# Autodesk Inventor assembly: Assembly6
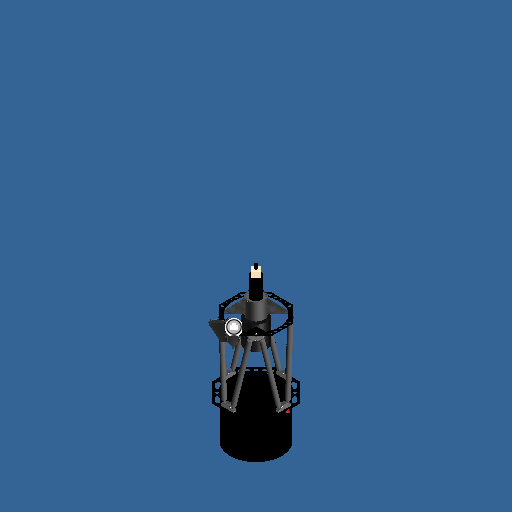
[picture p0: Inventor's stored thumbnail of the model, 512x512]
Saved by Autodesk Inventor 2026.2 (Build 302298000, 298)
## iProperties
Created: 2025-12-09
Part Number: Assembly6
Document SubType Name: Assembly
Designer: Thoma
Mass: 27295.5 g
Surface Area: 25498 cm^2
Volume: 10830.6 cm^3
Density: 2.52023 g/cm^3
Author: Thoma
## Documents named in this file (32)
- C:\Users\Thoma\OneDrive\Desktop\dir\telescope_cover\main\version_2\Main_v4.iam
- C:\Users\Thoma\OneDrive\Desktop\dir\telescope_cover\telescope\version_3\Telescope_End.ipt
- C:\Users\Thoma\OneDrive\Desktop\dir\telescope_cover\telescope\version_3\Triangle.ipt
- C:\Users\Thoma\OneDrive\Desktop\dir\telescope_cover\telescope\version_3\Triangle_Bracket_Top.ipt
- C:\Users\Thoma\OneDrive\Desktop\dir\telescope_cover\telescope\version_3\Carbon_Fibre.ipt
- C:\Users\Thoma\OneDrive\Desktop\dir\telescope_cover\telescope\version_3\5mm Screw.ipt
- C:\Users\Thoma\OneDrive\Desktop\dir\telescope_cover\telescope\version_3\35mm_bolt.ipt
- C:\Users\Thoma\OneDrive\Desktop\dir\telescope_cover\telescope\version_3\Triangle_Bracket_Bottom_MIR.ipt
- C:\Users\Thoma\OneDrive\Desktop\dir\telescope_cover\telescope\version_3\Telescope_Base.ipt
- C:\Users\Thoma\OneDrive\Desktop\dir\telescope_cover\telescope\version_3\Full_shaft_Simplify_3.ipt
- C:\Users\Thoma\OneDrive\Desktop\dir\telescope_cover\telescope\version_3\30mm_bolt.ipt
- C:\Users\Thoma\OneDrive\Desktop\dir\telescope_cover\telescope\version_3\Baffle.ipt
- C:\Users\Thoma\OneDrive\Desktop\dir\telescope_cover\telescope\version_3\Bottom_End_Top.ipt
- C:\Users\Thoma\OneDrive\Desktop\dir\telescope_cover\telescope\version_3\Laser.ipt
- C:\Users\Thoma\OneDrive\Desktop\dir\telescope_cover\cover\central_cover_v1.ipt
- C:\Users\Thoma\OneDrive\Desktop\dir\telescope_cover\cover\base_plate_v11.ipt
- C:\Users\Thoma\OneDrive\Desktop\dir\telescope_cover\cover\base_plate_bottom_v5.ipt
- C:\Users\Thoma\OneDrive\Documents\Inventor\Content Center Files\R2026\en-US\ISO 7089\ISO 7089 - 4 - 140 HV(1).ipt
- C:\Users\Thoma\OneDrive\Documents\Inventor\Content Center Files\R2026\en-US\ISO 4762(2)\ISO 4762 - M4 x 25ISO.ipt
- C:\Users\Thoma\OneDrive\Documents\Inventor\Content Center Files\R2026\en-US\ISO 4035(2)\ISO 4035 - M4 - ISO.ipt
- C:\Users\Thoma\OneDrive\Desktop\dir\telescope_cover\servo\DSS-M15S Servo.ipt
- C:\Users\Thoma\OneDrive\Documents\Inventor\Content Center Files\R2026\en-US\ISO 4762(2)\ISO 4762 - M4 x 16ISO.ipt
- C:\Users\Thoma\OneDrive\Desktop\dir\telescope_cover\cover\pawn_v3.ipt
- C:\Users\Thoma\OneDrive\Documents\Inventor\Content Center Files\R2026\en-US\DIN 6796\DIN 6796 - 2.ipt
- C:\Users\Thoma\OneDrive\Documents\Inventor\Content Center Files\R2026\en-US\DIN 912\DIN 912 - M2 x 0.4 x 8 x 7.ipt
- C:\Users\Thoma\OneDrive\Documents\Inventor\Content Center Files\R2026\en-US\DIN 912\DIN 912 - M2 x 0.4 x 5 x 4.ipt
- C:\Users\Thoma\OneDrive\Desktop\dir\telescope_cover\cover\rod_v11.ipt
- C:\Users\Thoma\OneDrive\Documents\Inventor\Content Center Files\R2026\en-US\ISO 7092\ISO 7092 - ST 4 - 140 HV.ipt
- C:\Users\Thoma\OneDrive\Desktop\dir\telescope_cover\cover\Cover_Upper_v5.ipt
- C:\Users\Thoma\OneDrive\Desktop\dir\telescope_cover\cover\4mm_washer_1mm.ipt
- C:\Users\Thoma\OneDrive\Documents\Inventor\Content Center Files\R2026\en-US\ISO 4762(2)\ISO 4762 - M4 x 20ISO.ipt
- C:\Users\Thoma\OneDrive\Desktop\dir\telescope_cover\servo\Limit Switch v3\Limit Switch v3\Limit Switch v3.ipt
## Components (98 placed, 31 different names)
1. base_plate_v11:1 — Mate:229, Angle:85, Mate:230, Mate:231, Mate:233, Mate:234, Mate:239, Mate:240, Mate:241, Angle:88, Mate:243, Mate:244, Mate:245, Angle:91, Mate:247, Mate:248, Mate:249, Angle:92, Mate:262, Mate:263, Mate:264, Mate:271, Mate:272, Mate:273, Mate:274, Mate:275, Mate:276, Mate:277, Mate:278, Mate:282, Mate:307, Mate:308, Mate:309, Mate:310, Mate:312, Mate:314
2. base_plate_bottom_v5:1 — Mate:232, Mate:233, Mate:234, Mate:242, Angle:89, Mate:246, Angle:90, Mate:250, Flush:227, Flush:228, Angle:93
3. ISO 7089 4:2 — Mate:239, Mate:240, Insert:2
4. ISO 4762 M4 x 25:1 — Insert:2, Angle:88
5. ISO 4035 M4:1 — Mate:241, Mate:242, Angle:89
6. ISO 7089 4:3 — Mate:243, Mate:244, Insert:3
7. ISO 4762 M4 x 16:1 — Insert:3, Angle:91
8. ISO 4035 M4:2 — Mate:245, Mate:246, Angle:90
9. ISO 7089 4:4 — Mate:247, Mate:248, Insert:4
10. ISO 4762 M4 x 16:2 — Insert:4
11. ISO 4035 M4:3 — Mate:249, Mate:250, Angle:93
12. pawn_v3:1 — Angle:92, Mate:281, Mate:282, Mate:311, Mate:313
13. DSS-M15S Servo:1 — Mate:262, Mate:263, Mate:264, Mate:279, Mate:280
14. DIN 6796 2:1 — Mate:271, Mate:272, Insert:6
15. DIN 912 - replaced by DIN EN ISO 4762 M2 x 8:1 — Insert:6
16. DIN 6796 2:2 — Mate:273, Mate:274, Insert:7
17. DIN 912 - replaced by DIN EN ISO 4762 M2 x 5:1 — Insert:7
18. DIN 6796 2:3 — Mate:275, Mate:276, Insert:8
19. DIN 912 - replaced by DIN EN ISO 4762 M2 x 8:2 — Insert:8
20. DIN 6796 2:4 — Mate:277, Mate:278, Insert:9
21. DIN 912 - replaced by DIN EN ISO 4762 M2 x 8:3 — Insert:9
22. rod_v11:1 — Mate:279, Mate:280, Mate:281, Mate:287, Mate:288, Tangent:34, Mate:289, Mate:290, Mate:291, Mate:292, Mate:293, Mate:294, Mate:295, Mate:297, Mate:298, Mate:299, Mate:301, Mate:302, Mate:303, Mate:305, Mate:306, Mate:315
23. Cover_Upper_v5:1 — Mate:287, Mate:288, Tangent:34, Mate:296, Mate:300, Mate:304
24. 4mm_washer_1mm:1 — Mate:289, Mate:294
25. 4mm_washer_1mm:2 — Mate:290, Mate:293
26. 4mm_washer_1mm:3 — Mate:291, Mate:292
27. ISO 7092 ST 4 - 140 HV:3 — Mate:295, Mate:296, Insert:12
28. ISO 4762 M4 x 16:3 — Insert:12
29. ISO 7092 ST 4 - 140 HV:4 — Mate:297, Mate:298, Insert:13
30. ISO 4035 M4:5 — Insert:13
31. ISO 7092 ST 4 - 140 HV:5 — Mate:299, Mate:300, Insert:14
32. ISO 4762 M4 x 16:4 — Insert:14
33. ISO 7092 ST 4 - 140 HV:6 — Mate:301, Mate:302, Insert:15
34. ISO 4035 M4:6 — Insert:15
35. ISO 7092 ST 4 - 140 HV:7 — Mate:303, Mate:304, Insert:16
36. ISO 4762 M4 x 16:5 — Insert:16
37. ISO 7092 ST 4 - 140 HV:8 — Mate:305, Mate:306, Insert:17
38. ISO 4035 M4:7 — Insert:17
39. ISO 4762 M4 x 20:1 — Mate:307, Mate:308
40. ISO 4035 M4:8 — Mate:309, Mate:310
41. ISO 4762 M4 x 20:2 — Mate:311, Mate:312
42. ISO 4035 M4:9 — Mate:313, Mate:314
43. Limit Switch v3:1 — Tangent:35
44. Limit Switch v3:2 — Flush:227, Flush:228, Mate:315
45. Laser:2 — Mate:214, Flush:220, Flush:221
46. Laser:1 — Mate:215, Flush:218, Flush:219
47. Baffle:1 — Mate:83
48. Carbon_Fibre:1 — Mate:7, Mate:11, Flush:1, Mate:12, Mate:13, Mate:14, Mate:15, Mate:62, Mate:83, Mate:92, Mate:93, Mate:96, Mate:97, Mate:98, Mate:100, Mate:123, Mate:124, Mate:125, Mate:213, Mate:220, Angle:84, Flush:223, Flush:224, Flush:225, Flush:226
49. Telescope_Base:1 — Mate:62, Angle:31, Mate:89, Mate:90, Angle:40, Mate:108, Mate:109, Angle:48, Mate:110, Mate:111, Angle:49, Mate:112, Mate:113, Angle:50, Mate:214, Mate:215, Flush:218, Flush:221
50. Telescope_End:1 — Mate:1, Mate:2, Angle:2, Mate:7, Mate:54, Mate:55, Angle:26, Angle:31, Mate:86, Mate:88, Mate:91, Angle:41, Mate:101, Angle:45, Angle:46, Mate:114, Mate:115, Angle:51, Mate:116, Mate:117, Angle:52, Mate:118, Mate:119, Angle:53, Mate:229, Angle:85, Mate:230, Mate:231, Mate:232
51. 30mm_bolt:9 — Mate:217, Mate:218, Angle:83
52. 30mm_bolt:10 — Mate:216, Mate:219, Angle:82
53. Triangle_Bracket_Top:5 — Mate:116, Mate:117, Angle:52, Mate:129, Flush:110, Angle:60
54. Triangle_Bracket_Top:4 — Mate:101, Angle:45, Angle:46, Mate:104, Mate:105, Mate:106, Flush:103, Angle:47
55. Triangle_Bracket_Top:3 — Mate:86, Mate:88, Mate:94, Angle:54, Angle:55, Mate:122, Flush:106, Angle:56
56. Triangle_Bracket_Top:1 — Mate:1, Mate:2, Angle:2, Mate:8, Mate:9, Angle:4, Mate:47, Angle:22, Mate:58
57. 5mm Screw:14 — Mate:220, Flush:222, Angle:84
58. Triangle:1 — Mate:8, Mate:9, Angle:4, Mate:11, Flush:1, Angle:5, Angle:6, Mate:46, Mate:222, Mate:223
59. Triangle:5 — Mate:92, Mate:93, Mate:94, Mate:128, Flush:109, Angle:59, Flush:181, Angle:81, Mate:225, Mate:227
60. Triangle:6 — Mate:96, Mate:97, Mate:98, Flush:102, Angle:44, Mate:104, Mate:105, Flush:222, Mate:221, Mate:228
61. Triangle:7 — Mate:123, Mate:124, Mate:125, Mate:126, Flush:107, Angle:57, Mate:127, Flush:108, Angle:58, Mate:224, Mate:226
62. 35mm_bolt:6 — Mate:122, Flush:106, Angle:56
63. 35mm_bolt:7 — Mate:129, Flush:110, Angle:60
64. 35mm_bolt:4 — Mate:46, Mate:47, Angle:22
65. 35mm_bolt:5 — Mate:106, Flush:103, Angle:47
66. 5mm Screw:9 — Mate:100, Flush:102, Angle:44
67. 5mm Screw:13 — Mate:213, Flush:181, Angle:81
68. 5mm Screw:10 — Mate:126, Flush:107, Angle:57
69. 5mm Screw:2 — Mate:14, Mate:15, Angle:6
70. 5mm Screw:1 — Mate:12, Mate:13, Angle:5
71. 5mm Screw:11 — Mate:127, Flush:108, Angle:58
72. 5mm Screw:12 — Mate:128, Flush:109, Angle:59
73. Full_shaft_Simplify_3:1
74. Full_shaft_Simplify_3:2 — Tangent:26
75. Full_shaft_Simplify_3:3
76. Full_shaft_Simplify_3:4
77. Full_shaft_Simplify_3:5
78. Full_shaft_Simplify_3:6
79. Full_shaft_Simplify_3:7
80. Full_shaft_Simplify_3:8 — Tangent:31, Tangent:33
81. 30mm_bolt:7 — Mate:120, Flush:104, Angle:54
82. 30mm_bolt:1 — Mate:121, Flush:105, Angle:55
83. 30mm_bolt:8 — Mate:80, Flush:13, Angle:39
84. 30mm_bolt:6 — Mate:78, Flush:11, Angle:37
85. 30mm_bolt:3 — Mate:79, Flush:12, Angle:38
86. 30mm_bolt:2 — Mate:77, Flush:10, Angle:36
87. Triangle_Bracket_Bottom_MIR:4 — Mate:118, Mate:119, Angle:53, Mate:216, Mate:217, Mate:218, Mate:219, Angle:82, Angle:83
88. Triangle_Bracket_Bottom_MIR:3 — Mate:114, Mate:115, Angle:51, Mate:120, Flush:104, Mate:121, Flush:105
89. Triangle_Bracket_Bottom_MIR:2 — Mate:55, Mate:58, Angle:26, Mate:77, Flush:10, Angle:36, Mate:78, Flush:11, Angle:37, Tangent:31
90. Triangle_Bracket_Bottom_MIR:1 — Mate:54, Mate:79, Flush:12, Angle:38, Mate:80, Flush:13, Angle:39, Mate:91, Angle:41
91. Bottom_End_Top:4 — Mate:112, Mate:113, Angle:50, Tangent:26, Tangent:33
92. Bottom_End_Top:3 — Mate:110, Mate:111, Angle:49, Flush:219
93. Bottom_End_Top:2 — Mate:108, Mate:109, Angle:48
94. Bottom_End_Top:1 — Mate:89, Mate:90, Angle:40, Flush:220
95. central_cover_v1:1 — Mate:221, Mate:222, Flush:223, Tangent:35
96. central_cover_v1:2 — Mate:223, Mate:224, Flush:224
97. central_cover_v1:3 — Mate:225, Mate:226, Flush:225
98. central_cover_v1:4 — Mate:227, Mate:228, Flush:226
## Relationships (222: Mate 137, Angle 41, Flush 26, Insert 13, Tangent 5)
- Mate:1: Telescope_End:1 ↔ Triangle_Bracket_Top:1
- Mate:2: Telescope_End:1 ↔ Triangle_Bracket_Top:1
- Angle:2 (0 deg): Telescope_End:1 ↔ Triangle_Bracket_Top:1
- Mate:7: Carbon_Fibre:1 ↔ Telescope_End:1
- Mate:8: Triangle_Bracket_Top:1 ↔ Triangle:1
- Mate:9: Triangle_Bracket_Top:1 ↔ Triangle:1
- Angle:4 (0 deg): Triangle_Bracket_Top:1 ↔ Triangle:1
- Mate:11: Carbon_Fibre:1 ↔ Triangle:1
- Flush:1: Carbon_Fibre:1 ↔ Triangle:1
- Mate:12: Carbon_Fibre:1 ↔ 5mm Screw:1
- Mate:13: Carbon_Fibre:1 ↔ 5mm Screw:1
- Angle:5 (0 deg): Triangle:1 ↔ 5mm Screw:1
- Mate:14: Carbon_Fibre:1 ↔ 5mm Screw:2
- Mate:15: Carbon_Fibre:1 ↔ 5mm Screw:2
- Angle:6 (0 deg): Triangle:1 ↔ 5mm Screw:2
- Mate:46: Triangle:1 ↔ 35mm_bolt:4
- Mate:47: Triangle_Bracket_Top:1 ↔ 35mm_bolt:4
- Angle:22 (0 deg): Triangle_Bracket_Top:1 ↔ 35mm_bolt:4
- Mate:54: Telescope_End:1 ↔ Triangle_Bracket_Bottom_MIR:1
- Mate:55: Telescope_End:1 ↔ Triangle_Bracket_Bottom_MIR:2
- Mate:58: Triangle_Bracket_Top:1 ↔ Triangle_Bracket_Bottom_MIR:2
- Angle:26 (0 deg): Telescope_End:1 ↔ Triangle_Bracket_Bottom_MIR:2
- Mate:62: Carbon_Fibre:1 ↔ Telescope_Base:1
- Angle:31 (0 deg): Telescope_Base:1 ↔ Telescope_End:1
- Mate:77: 30mm_bolt:2 ↔ Triangle_Bracket_Bottom_MIR:2
- Flush:10: 30mm_bolt:2 ↔ Triangle_Bracket_Bottom_MIR:2
- Angle:36 (0 deg): 30mm_bolt:2 ↔ Triangle_Bracket_Bottom_MIR:2
- Mate:78: 30mm_bolt:6 ↔ Triangle_Bracket_Bottom_MIR:2
- Flush:11: 30mm_bolt:6 ↔ Triangle_Bracket_Bottom_MIR:2
- Angle:37 (0 deg): 30mm_bolt:6 ↔ Triangle_Bracket_Bottom_MIR:2
- Mate:79: 30mm_bolt:3 ↔ Triangle_Bracket_Bottom_MIR:1
- Flush:12: 30mm_bolt:3 ↔ Triangle_Bracket_Bottom_MIR:1
- Angle:38 (0 deg): 30mm_bolt:3 ↔ Triangle_Bracket_Bottom_MIR:1
- Mate:80: 30mm_bolt:8 ↔ Triangle_Bracket_Bottom_MIR:1
- Flush:13: 30mm_bolt:8 ↔ Triangle_Bracket_Bottom_MIR:1
- Angle:39 (0 deg): 30mm_bolt:8 ↔ Triangle_Bracket_Bottom_MIR:1
- Mate:83: Baffle:1 ↔ Carbon_Fibre:1
- Mate:86: Telescope_End:1 ↔ Triangle_Bracket_Top:3
- Mate:88: Telescope_End:1 ↔ Triangle_Bracket_Top:3
- Mate:89: Telescope_Base:1 ↔ Bottom_End_Top:1
- Mate:90: Telescope_Base:1 ↔ Bottom_End_Top:1
- Angle:40 (0 deg): Telescope_Base:1 ↔ Bottom_End_Top:1
- Mate:91: Telescope_End:1 ↔ Triangle_Bracket_Bottom_MIR:1
- Angle:41 (0 deg): Telescope_End:1 ↔ Triangle_Bracket_Bottom_MIR:1
- Mate:92: Carbon_Fibre:1 ↔ Triangle:5
- Mate:93: Carbon_Fibre:1 ↔ Triangle:5
- Mate:94: Triangle_Bracket_Top:3 ↔ Triangle:5
- Mate:96: Carbon_Fibre:1 ↔ Triangle:6
- Mate:97: Carbon_Fibre:1 ↔ Triangle:6
- Mate:98: Carbon_Fibre:1 ↔ Triangle:6
- Mate:100: Carbon_Fibre:1 ↔ 5mm Screw:9
- Flush:102: Triangle:6 ↔ 5mm Screw:9
- Angle:44 (0 deg): Triangle:6 ↔ 5mm Screw:9
- Mate:101: Telescope_End:1 ↔ Triangle_Bracket_Top:4
- Angle:45 (0 deg): Telescope_End:1 ↔ Triangle_Bracket_Top:4
- Angle:46 (0 deg): Telescope_End:1 ↔ Triangle_Bracket_Top:4
- Mate:104: Triangle_Bracket_Top:4 ↔ Triangle:6
- Mate:105: Triangle_Bracket_Top:4 ↔ Triangle:6
- Mate:106: Triangle_Bracket_Top:4 ↔ 35mm_bolt:5
- Flush:103: Triangle_Bracket_Top:4 ↔ 35mm_bolt:5
- Angle:47 (0 deg): Triangle_Bracket_Top:4 ↔ 35mm_bolt:5
- Mate:108: Telescope_Base:1 ↔ Bottom_End_Top:2
- Mate:109: Telescope_Base:1 ↔ Bottom_End_Top:2
- Angle:48 (0 deg): Telescope_Base:1 ↔ Bottom_End_Top:2
- Mate:110: Telescope_Base:1 ↔ Bottom_End_Top:3
- Mate:111: Telescope_Base:1 ↔ Bottom_End_Top:3
- Angle:49 (0 deg): Telescope_Base:1 ↔ Bottom_End_Top:3
- Mate:112: Telescope_Base:1 ↔ Bottom_End_Top:4
- Mate:113: Telescope_Base:1 ↔ Bottom_End_Top:4
- Angle:50 (0 deg): Telescope_Base:1 ↔ Bottom_End_Top:4
- Mate:114: Telescope_End:1 ↔ Triangle_Bracket_Bottom_MIR:3
- Mate:115: Telescope_End:1 ↔ Triangle_Bracket_Bottom_MIR:3
- Angle:51 (0 deg): Telescope_End:1 ↔ Triangle_Bracket_Bottom_MIR:3
- Mate:116: Telescope_End:1 ↔ Triangle_Bracket_Top:5
- Mate:117: Telescope_End:1 ↔ Triangle_Bracket_Top:5
- Angle:52 (0 deg): Telescope_End:1 ↔ Triangle_Bracket_Top:5
- Mate:118: Telescope_End:1 ↔ Triangle_Bracket_Bottom_MIR:4
- Mate:119: Telescope_End:1 ↔ Triangle_Bracket_Bottom_MIR:4
- Angle:53 (0 deg): Telescope_End:1 ↔ Triangle_Bracket_Bottom_MIR:4
- Mate:120: 30mm_bolt:7 ↔ Triangle_Bracket_Bottom_MIR:3
- Flush:104: 30mm_bolt:7 ↔ Triangle_Bracket_Bottom_MIR:3
- Angle:54 (0 deg): Triangle_Bracket_Top:3 ↔ 30mm_bolt:7
- Mate:121: 30mm_bolt:1 ↔ Triangle_Bracket_Bottom_MIR:3
- Flush:105: 30mm_bolt:1 ↔ Triangle_Bracket_Bottom_MIR:3
- Angle:55 (0 deg): Triangle_Bracket_Top:3 ↔ 30mm_bolt:1
- Mate:122: Triangle_Bracket_Top:3 ↔ 35mm_bolt:6
- Flush:106: Triangle_Bracket_Top:3 ↔ 35mm_bolt:6
- Angle:56 (0 deg): Triangle_Bracket_Top:3 ↔ 35mm_bolt:6
- Mate:123: Carbon_Fibre:1 ↔ Triangle:7
- Mate:124: Carbon_Fibre:1 ↔ Triangle:7
- Mate:125: Carbon_Fibre:1 ↔ Triangle:7
- Mate:126: Triangle:7 ↔ 5mm Screw:10
- Flush:107: Triangle:7 ↔ 5mm Screw:10
- Angle:57 (0 deg): Triangle:7 ↔ 5mm Screw:10
- Mate:127: Triangle:7 ↔ 5mm Screw:11
- Flush:108: Triangle:7 ↔ 5mm Screw:11
- Angle:58 (0 deg): Triangle:7 ↔ 5mm Screw:11
- Mate:128: Triangle:5 ↔ 5mm Screw:12
- Flush:109: Triangle:5 ↔ 5mm Screw:12
- Angle:59 (0 deg): Triangle:5 ↔ 5mm Screw:12
- Mate:129: Triangle_Bracket_Top:5 ↔ 35mm_bolt:7
- Flush:110: Triangle_Bracket_Top:5 ↔ 35mm_bolt:7
- Angle:60 (0 deg): Triangle_Bracket_Top:5 ↔ 35mm_bolt:7
- Mate:213: Carbon_Fibre:1 ↔ 5mm Screw:13
- Flush:181: Triangle:5 ↔ 5mm Screw:13
- Angle:81 (0 deg): Triangle:5 ↔ 5mm Screw:13
- Mate:214: Laser:2 ↔ Telescope_Base:1
- Mate:215: Laser:1 ↔ Telescope_Base:1
- Flush:218: Laser:1 ↔ Telescope_Base:1
- Flush:219 (39.316 mm): Laser:1 ↔ Bottom_End_Top:3
- Flush:220 (39.316 mm): Laser:2 ↔ Bottom_End_Top:1
- Flush:221: Laser:2 ↔ Telescope_Base:1
- Tangent:26: Full_shaft_Simplify_3:2 ↔ Bottom_End_Top:4
- Tangent:31: Full_shaft_Simplify_3:8 ↔ Triangle_Bracket_Bottom_MIR:2
- Tangent:33: Full_shaft_Simplify_3:8 ↔ Bottom_End_Top:4
- Mate:216: 30mm_bolt:10 ↔ Triangle_Bracket_Bottom_MIR:4
- Mate:217: 30mm_bolt:9 ↔ Triangle_Bracket_Bottom_MIR:4
- Mate:218: 30mm_bolt:9 ↔ Triangle_Bracket_Bottom_MIR:4
- Mate:219: 30mm_bolt:10 ↔ Triangle_Bracket_Bottom_MIR:4
- Angle:82 (0 deg): 30mm_bolt:10 ↔ Triangle_Bracket_Bottom_MIR:4
- Angle:83 (0 deg): 30mm_bolt:9 ↔ Triangle_Bracket_Bottom_MIR:4
- Mate:220: Carbon_Fibre:1 ↔ 5mm Screw:14
- Flush:222: 5mm Screw:14 ↔ Triangle:6
- Angle:84 (0 deg): Carbon_Fibre:1 ↔ 5mm Screw:14
- Mate:221: Triangle:6 ↔ central_cover_v1:1
- Mate:222: Triangle:1 ↔ central_cover_v1:1
- Flush:223: Carbon_Fibre:1 ↔ central_cover_v1:1
- Mate:223: Triangle:1 ↔ central_cover_v1:2
- Mate:224: Triangle:7 ↔ central_cover_v1:2
- Flush:224: Carbon_Fibre:1 ↔ central_cover_v1:2
- Mate:225: Triangle:5 ↔ central_cover_v1:3
- Mate:226: Triangle:7 ↔ central_cover_v1:3
- Flush:225: Carbon_Fibre:1 ↔ central_cover_v1:3
- Mate:227: Triangle:5 ↔ central_cover_v1:4
- Mate:228: Triangle:6 ↔ central_cover_v1:4
- Flush:226: Carbon_Fibre:1 ↔ central_cover_v1:4
- Mate:229: base_plate_v11:1 ↔ Telescope_End:1
- Angle:85 (0 deg): base_plate_v11:1 ↔ Telescope_End:1
- Mate:230: base_plate_v11:1 ↔ Telescope_End:1
- Mate:231: base_plate_v11:1 ↔ Telescope_End:1
- Mate:232: base_plate_bottom_v5:1 ↔ Telescope_End:1
- Mate:233: base_plate_v11:1 ↔ base_plate_bottom_v5:1
- Mate:234: base_plate_v11:1 ↔ base_plate_bottom_v5:1
- Mate:239: base_plate_v11:1 ↔ ISO 7089 4:2
- Mate:240: base_plate_v11:1 ↔ ISO 7089 4:2
- Insert:2: ISO 7089 4:2 ↔ ISO 4762 M4 x 25:1
- Mate:241: base_plate_v11:1 ↔ ISO 4035 M4:1
- Mate:242: base_plate_bottom_v5:1 ↔ ISO 4035 M4:1
- Angle:88 (0 deg): base_plate_v11:1 ↔ ISO 4762 M4 x 25:1
- Angle:89 (0 deg): base_plate_bottom_v5:1 ↔ ISO 4035 M4:1
- Mate:243: base_plate_v11:1 ↔ ISO 7089 4:3
- Mate:244: base_plate_v11:1 ↔ ISO 7089 4:3
- Insert:3: ISO 7089 4:3 ↔ ISO 4762 M4 x 16:1
- Mate:245: base_plate_v11:1 ↔ ISO 4035 M4:2
- Mate:246: base_plate_bottom_v5:1 ↔ ISO 4035 M4:2
- Angle:90 (0 deg): base_plate_bottom_v5:1 ↔ ISO 4035 M4:2
- Angle:91 (0 deg): base_plate_v11:1 ↔ ISO 4762 M4 x 16:1
- Mate:247: base_plate_v11:1 ↔ ISO 7089 4:4
- Mate:248: base_plate_v11:1 ↔ ISO 7089 4:4
- Insert:4: ISO 7089 4:4 ↔ ISO 4762 M4 x 16:2
- Mate:249: base_plate_v11:1 ↔ ISO 4035 M4:3
- Mate:250: base_plate_bottom_v5:1 ↔ ISO 4035 M4:3
- Angle:92 (0 deg): base_plate_v11:1 ↔ pawn_v3:1
- Mate:262: base_plate_v11:1 ↔ DSS-M15S Servo:1
- Mate:263 (1.1 mm): base_plate_v11:1 ↔ DSS-M15S Servo:1
- Mate:264: base_plate_v11:1 ↔ DSS-M15S Servo:1
- Mate:271: base_plate_v11:1 ↔ DIN 6796 2:1
- Mate:272: base_plate_v11:1 ↔ DIN 6796 2:1
- Insert:6: DIN 6796 2:1 ↔ DIN 912 - replaced by DIN EN ISO 4762 M2 x 8:1
- Mate:273: base_plate_v11:1 ↔ DIN 6796 2:2
- Mate:274: base_plate_v11:1 ↔ DIN 6796 2:2
- Insert:7: DIN 6796 2:2 ↔ DIN 912 - replaced by DIN EN ISO 4762 M2 x 5:1
- Mate:275: base_plate_v11:1 ↔ DIN 6796 2:3
- Mate:276: base_plate_v11:1 ↔ DIN 6796 2:3
- Insert:8: DIN 6796 2:3 ↔ DIN 912 - replaced by DIN EN ISO 4762 M2 x 8:2
- Mate:277: base_plate_v11:1 ↔ DIN 6796 2:4
- Mate:278: base_plate_v11:1 ↔ DIN 6796 2:4
- Insert:9: DIN 6796 2:4 ↔ DIN 912 - replaced by DIN EN ISO 4762 M2 x 8:3
- Mate:279: DSS-M15S Servo:1 ↔ rod_v11:1
- Mate:280: DSS-M15S Servo:1 ↔ rod_v11:1
- Mate:281: pawn_v3:1 ↔ rod_v11:1
- Mate:282 (0.4 mm): base_plate_v11:1 ↔ pawn_v3:1
- Mate:287: rod_v11:1 ↔ Cover_Upper_v5:1
- Mate:288: rod_v11:1 ↔ Cover_Upper_v5:1
- Tangent:34 (-1 mm): rod_v11:1 ↔ Cover_Upper_v5:1
- Mate:289: rod_v11:1 ↔ 4mm_washer_1mm:1
- Mate:290: rod_v11:1 ↔ 4mm_washer_1mm:2
- Mate:291: rod_v11:1 ↔ 4mm_washer_1mm:3
- Mate:292: rod_v11:1 ↔ 4mm_washer_1mm:3
- Mate:293: rod_v11:1 ↔ 4mm_washer_1mm:2
- Mate:294: rod_v11:1 ↔ 4mm_washer_1mm:1
- Mate:295: rod_v11:1 ↔ ISO 7092 ST 4 - 140 HV:3
- Mate:296: Cover_Upper_v5:1 ↔ ISO 7092 ST 4 - 140 HV:3
- Insert:12: ISO 7092 ST 4 - 140 HV:3 ↔ ISO 4762 M4 x 16:3
- Mate:297: rod_v11:1 ↔ ISO 7092 ST 4 - 140 HV:4
- Mate:298: rod_v11:1 ↔ ISO 7092 ST 4 - 140 HV:4
- Insert:13: ISO 7092 ST 4 - 140 HV:4 ↔ ISO 4035 M4:5
- Mate:299: rod_v11:1 ↔ ISO 7092 ST 4 - 140 HV:5
- Mate:300: Cover_Upper_v5:1 ↔ ISO 7092 ST 4 - 140 HV:5
- Insert:14: ISO 7092 ST 4 - 140 HV:5 ↔ ISO 4762 M4 x 16:4
- Mate:301: rod_v11:1 ↔ ISO 7092 ST 4 - 140 HV:6
- Mate:302: rod_v11:1 ↔ ISO 7092 ST 4 - 140 HV:6
- Insert:15: ISO 7092 ST 4 - 140 HV:6 ↔ ISO 4035 M4:6
- Mate:303: rod_v11:1 ↔ ISO 7092 ST 4 - 140 HV:7
- Mate:304: Cover_Upper_v5:1 ↔ ISO 7092 ST 4 - 140 HV:7
- Insert:16: ISO 7092 ST 4 - 140 HV:7 ↔ ISO 4762 M4 x 16:5
- Mate:305: rod_v11:1 ↔ ISO 7092 ST 4 - 140 HV:8
- Mate:306: rod_v11:1 ↔ ISO 7092 ST 4 - 140 HV:8
- Insert:17: ISO 7092 ST 4 - 140 HV:8 ↔ ISO 4035 M4:7
- Mate:307: base_plate_v11:1 ↔ ISO 4762 M4 x 20:1
- Mate:308: base_plate_v11:1 ↔ ISO 4762 M4 x 20:1
- Mate:309: base_plate_v11:1 ↔ ISO 4035 M4:8
- Mate:310: base_plate_v11:1 ↔ ISO 4035 M4:8
- Mate:311: pawn_v3:1 ↔ ISO 4762 M4 x 20:2
- Mate:312: base_plate_v11:1 ↔ ISO 4762 M4 x 20:2
- Mate:313: pawn_v3:1 ↔ ISO 4035 M4:9
- Mate:314: base_plate_v11:1 ↔ ISO 4035 M4:9
- Tangent:35: Limit Switch v3:1 ↔ central_cover_v1:1
- Flush:227 (-10 mm): base_plate_bottom_v5:1 ↔ Limit Switch v3:2
- Flush:228: base_plate_bottom_v5:1 ↔ Limit Switch v3:2
- Mate:315: rod_v11:1 ↔ Limit Switch v3:2
- Angle:93 (0 deg): base_plate_bottom_v5:1 ↔ ISO 4035 M4:3
